# Autodesk Inventor assembly: Orangatang_Kegel_w_Pulley
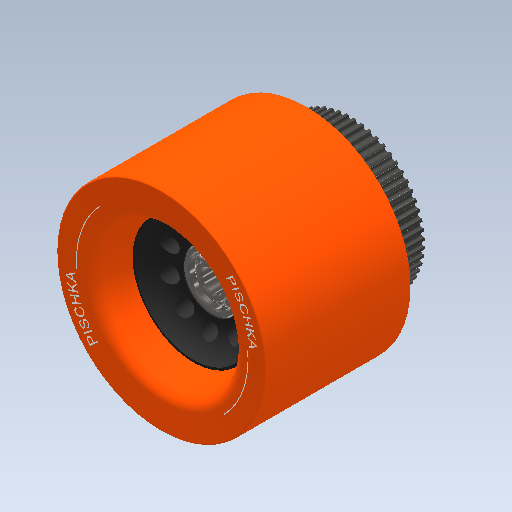
[picture p0: Inventor's stored thumbnail of the model, 512x512]
Saved by Autodesk Inventor 2020.1 (Build 241239000, 239)
## iProperties
Created: 2018-07-26
Part Number: Orangatang_Kegel_w_Pulley
Document SubType Name: Assembly
Designer: Tobias
Mass: 403.838 g
Surface Area: 619.162 cm^2
Volume: 255.202 cm^3
Density: 1.58243 g/cm^3
Author: Tobias
## Documents named in this file (6)
- D:\OMG\E-Board\CAD\Inventor\Trucks\Orangatang Kegel\Orangatang_Kegel_w_Pulley.iam
- D:\OMG\E-Board\CAD\Inventor\Trucks\Orangatang Kegel\Kegel_core.ipt
- D:\OMG\E-Board\CAD\Inventor\Trucks\Orangatang Kegel\Kegel_urethane.ipt
- D:\OMG\E-Board\CAD\Inventor\Trucks\spacer.ipt
- D:\OMG\E-Board\CAD\Inventor\Trucks\Bearings\bearing_abec7.iam
- D:\OMG\E-Board\CAD\Inventor\Mechanical Components\Wheel Pulley\Orangatang Kegel Adapter - z60.ipt
## Components (6 placed, 5 different names)
1. Kegel_core:1 — Mate:1, Flush:3, Flush:4, Mate:4, Mate:5, Mate:6, Insert:1, Insert:3, Insert:4
2. Kegel_urethane:1 — Mate:4, Mate:5, Mate:6
3. spacer:1 — Insert:2
4. bearing_abec7:1 [sub-assembly] — Insert:1, Insert:2
5. bearing_abec7:2 [sub-assembly] — Insert:3
6. Orangatang Kegel Adapter:1 — Insert:4
## Relationships (10: Mate 4, Insert 4, Flush 2)
- Mate:1: Kegel_core:1
- Flush:3: Kegel_core:1
- Flush:4: Kegel_core:1
- Mate:4: Kegel_core:1 ↔ Kegel_urethane:1
- Mate:5: Kegel_core:1 ↔ Kegel_urethane:1
- Mate:6: Kegel_core:1 ↔ Kegel_urethane:1
- Insert:1: Kegel_core:1 ↔ bearing_abec7:1
- Insert:2: spacer:1 ↔ bearing_abec7:1
- Insert:3: Kegel_core:1 ↔ bearing_abec7:2
- Insert:4: Kegel_core:1 ↔ Orangatang Kegel Adapter:1
